# Autodesk Inventor assembly: 341-01
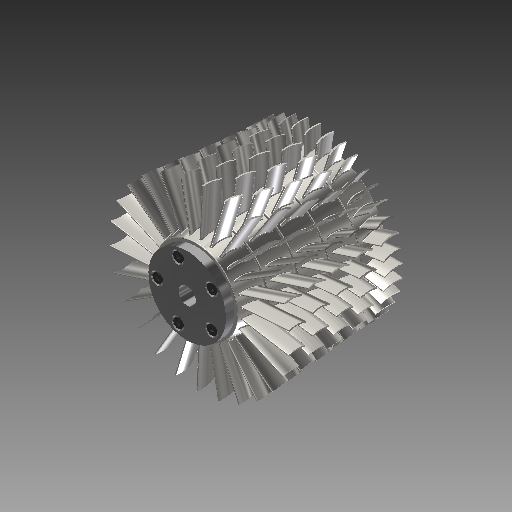
[picture p0: Inventor's stored thumbnail of the model, 512x512]
Saved by Autodesk Inventor 2019 (Build 230136000, 136)
## iProperties
Created: 2017-06-23
Part Number: 341-01
Document SubType Name: Assembly
Designer: t_crawk
Mass: 8279.77 g
Surface Area: 5762.84 cm^2
Volume: 1829.78 cm^3
Density: 4.52502 g/cm^3
Author: t_crawk
## Documents named in this file (11)
- C:\TEMP\Jet Engine Model\Workspace\Mid Compression Assembly.iam
- C:\TEMP\Jet Engine Model\Workspace\Mid Compression Shaft.ipt
- C:\TEMP\Jet Engine Model\Workspace\Compression Fan-1.ipt
- C:\TEMP\Jet Engine Model\Workspace\Mid Compression Link.ipt
- C:\TEMP\Jet Engine Model\Workspace\Front Compression Fan\Front Compression Fan-01.ipt
- C:\Users\t_crawk\Documents\Inventor\Sample Files\Jet Engine V2\Compression\Front Compression Fan.ipt
- C:\TEMP\Jet Engine Model\Workspace\Front Compression Fan\Front Compression Fan-02.ipt
- C:\TEMP\Jet Engine Model\Workspace\Front Compression Fan\Front Compression Fan-03.ipt
- C:\TEMP\Jet Engine Model\Workspace\Front Compression Fan\Front Compression Fan-04.ipt
- C:\TEMP\Jet Engine Model\Workspace\Front Compression Hub.ipt
- C:\TEMP\Jet Engine Model\Libraries\Content Center Files\en-US\ISO 10642(1)\ISO 10642 - M6 x  25.ipt
## Components (22 placed, 9 different names)
1. Mid Compression Shaft:1 — Flush:1, Flush:2, Flush:3, Insert:1, Insert:2, Insert:8
2. Compression Fan-1:1 — Insert:1, Mate:1, Insert:3
3. Front Compression Fan-01:1 — Insert:3, Mate:2, Insert:4
4. Front Compression Fan-02:2 — Insert:4, Mate:3, Insert:5
5. Front Compression Fan-03:3 — Mate:5, Insert:5, Insert:6
6. Front Compression Fan-04:4 — Insert:6, Mate:6, Insert:7
7. Front Compression Hub:1 — Insert:7, Mate:7, Insert:9
8. Mid Compression Link:1 — Insert:2, Mate:1, Mate:2, Mate:3, Mate:5, Mate:6
9. Mid Compression Link:2
10. Mid Compression Link:3
11. Mid Compression Link:4
12. Mid Compression Link:5 — Mate:7
13. ISO 10642 M6 x  25:1 — Insert:8
14. ISO 10642 M6 x  25:3
15. ISO 10642 M6 x  25:4
16. ISO 10642 M6 x  25:5
17. ISO 10642 M6 x  25:6
18. ISO 10642 M6 x  25:2 — Insert:9
19. ISO 10642 M6 x  25:7
20. ISO 10642 M6 x  25:8
21. ISO 10642 M6 x  25:9
22. ISO 10642 M6 x  25:10
## Component patterns: (5 elements, first: Mid Compression Link:1), (5 elements, first: ISO 10642 M6 x  25:1), (5 elements, first: ISO 10642 M6 x  25:2)
## Relationships (18: Insert 9, Mate 6, Flush 3)
- Flush:1: Mid Compression Shaft:1
- Flush:2: Mid Compression Shaft:1
- Flush:3: Mid Compression Shaft:1
- Insert:1: Mid Compression Shaft:1 ↔ Compression Fan-1:1
- Insert:2: Mid Compression Shaft:1 ↔ Mid Compression Link:1
- Mate:1: Compression Fan-1:1 ↔ Mid Compression Link:1
- Insert:3: Compression Fan-1:1 ↔ Front Compression Fan-01:1
- Mate:2: Front Compression Fan-01:1 ↔ Mid Compression Link:1
- Insert:4: Front Compression Fan-01:1 ↔ Front Compression Fan-02:2
- Mate:3: Front Compression Fan-02:2 ↔ Mid Compression Link:1
- Mate:5: Front Compression Fan-03:3 ↔ Mid Compression Link:1
- Insert:5: Front Compression Fan-02:2 ↔ Front Compression Fan-03:3
- Insert:6: Front Compression Fan-03:3 ↔ Front Compression Fan-04:4
- Mate:6: Front Compression Fan-04:4 ↔ Mid Compression Link:1
- Insert:7: Front Compression Fan-04:4 ↔ Front Compression Hub:1
- Mate:7: Front Compression Hub:1 ↔ Mid Compression Link:5
- Insert:8: Mid Compression Shaft:1 ↔ ISO 10642 M6 x  25:1
- Insert:9: Front Compression Hub:1 ↔ ISO 10642 M6 x  25:2
